# Autodesk Inventor assembly: FirstJoint
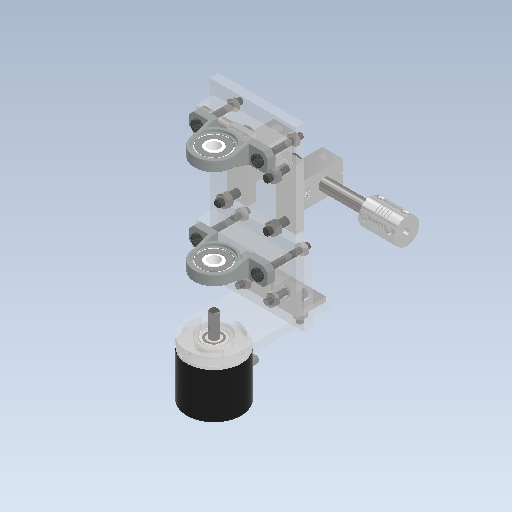
[picture p0: Inventor's stored thumbnail of the model, 512x512]
Saved by Autodesk Inventor 2021.1 (Build 251245010, 245A)
## iProperties
Created: 2023-10-30
Part Number: FirstJoint
Document SubType Name: Assembly
Designer: M
Mass: 466.393 g
Surface Area: 850.201 cm^2
Volume: 171.89 cm^3
Density: 2.71332 g/cm^3
Author: M
## Documents named in this file (17)
- F:\College\Semester_10\GP2\2DOF\2DOF_Hover\CAD\Workspaces\Workspace\FirstJoint.iam
- F:\College\Semester_10\GP2\2DOF\2DOF_Hover\CAD\Workspaces\Workspace\shaft.ipt
- F:\College\Semester_10\GP2\2DOF\2DOF_Hover\CAD\Workspaces\Workspace\Encoder.ipt
- F:\College\Semester_10\GP2\2DOF\2DOF_Hover\CAD\Workspaces\Workspace\KP008.ipt
- F:\College\Semester_10\GP2\2DOF\2DOF_Hover\CAD\Workspaces\Workspace\Holder Tube-R8.ipt
- F:\College\Semester_10\GP2\2DOF\2DOF_Hover\CAD\Workspaces\Workspace\interplate.ipt
- F:\College\Semester_10\GP2\2DOF\2DOF_Hover\CAD\Workspaces\Workspace\plateplummer.ipt
- F:\College\Semester_10\GP2\2DOF\2DOF_Hover\CAD\Workspaces\Workspace\plateencoder.ipt
- F:\College\Semester_10\GP2\2DOF\2DOF_Hover\CAD\Workspaces\Workspace\Joint1C_1.ipt
- F:\College\Semester_10\GP2\2DOF\2DOF_Hover\CAD\Workspaces\Workspace\2020RightAngle.ipt
- F:\College\Semester_10\GP2\2DOF\2DOF_Hover\CAD\Libraries\Content Center Files\en-US\ISO 4017(1)\ISO 4017 - M4 x 16 - ISO.ipt
- F:\College\Semester_10\GP2\2DOF\2DOF_Hover\CAD\Libraries\Content Center Files\en-US\ISO 4032(2)\ISO 4032 - M4 - ISO.ipt
- F:\College\Semester_10\GP2\2DOF\2DOF_Hover\CAD\Libraries\Content Center Files\en-US\ISO 7045  H\ISO 7045 - M5 x 20 - 4.8 - H - ISO.ipt
- F:\College\Semester_10\GP2\2DOF\2DOF_Hover\CAD\Libraries\Content Center Files\en-US\ISO 4032(2)\ISO 4032 - M5 - ISO.ipt
- F:\College\Semester_10\GP2\2DOF\2DOF_Hover\CAD\Libraries\Content Center Files\en-US\ISO 7045  H\ISO 7045 - M4 x 35 - 4.8 - H - ISO.ipt
- F:\College\Semester_10\GP2\2DOF\2DOF_Hover\CAD\Libraries\Content Center Files\en-US\ISO 7045  H\ISO 7045 - M4 x 30 - 4.8 - H - ISO.ipt
- F:\College\Semester_10\GP2\2DOF\2DOF_Hover\CAD\Workspaces\Workspace\Coupler_5x8.ipt
## Components (38 placed, 16 different names)
1. shaft:1 — Mate:81, Mate:82
2. Encoder:1 — Mate:17, Mate:23
3. KP008:1 — Mate:71, Mate:72, Mate:73, Mate:75, Mate:76
4. KP008:2 — Mate:18, Mate:63, Mate:64, Mate:65, Mate:67, Mate:68
5. Holder Tube-R8:1 — Mate:47, Mate:48, Mate:49, Mate:59, Mate:60
6. Holder Tube-R8:2 — Mate:51, Mate:52, Mate:55, Mate:56, Mate:79, Mate:80
7. interplate:1 — Flush:13, Mate:19, Mate:20, Mate:21, Mate:22, Angle:1, Mate:26, Mate:27, Mate:50, Mate:54, Mate:58, Mate:61, Mate:74, Mate:77
8. plateplummer:1 — Mate:19, Mate:20
9. plateplummer:2 — Mate:18, Mate:21, Mate:22
10. plateencoder:1 — Mate:26, Mate:27, Mate:28, Mate:29, Flush:14, Flush:15, Mate:39, Mate:41, Mate:42, Mate:43, Mate:45, Mate:66, Mate:70
11. Joint1C_1:1 — Mate:17, Mate:23, Angle:1, Mate:30, Flush:16, Flush:17, Mate:31, Mate:33, Mate:34, Mate:35, Mate:38
12. 2020RightAngle:1 — Mate:29, Flush:14, Mate:30, Flush:16, Mate:32, Mate:40
13. 2020RightAngle:2 — Mate:28, Flush:15, Flush:17, Mate:36, Mate:44
14. Coupler_5x8:1 — Mate:81, Mate:82
15. ISO 4017 M4 x 16:1 — Mate:31, Mate:32
16. ISO 4032 M4:1 — Mate:33, Mate:34
17. ISO 4017 M4 x 16:2 — Mate:35, Mate:36, Mate:37
18. ISO 4032 M4:2 — Mate:37, Mate:38
19. ISO 4017 M4 x 16:3 — Mate:39, Mate:40
20. ISO 4032 M4:3 — Mate:41, Mate:42
21. ISO 4017 M4 x 16:4 — Mate:43, Mate:44, Mate:46
22. ISO 4032 M4:4 — Mate:45, Mate:46
23. ISO 7045 H M5 x 20 - 4.8 - H:1 — Mate:47, Mate:48
24. ISO 4032 M5:1 — Mate:49, Mate:50
25. ISO 7045 H M5 x 20 - 4.8 - H:2 — Mate:55, Mate:56, Mate:57
26. ISO 4032 M5:2 — Mate:57, Mate:58
27. ISO 7045 H M5 x 20 - 4.8 - H:3 — Mate:59, Mate:60, Mate:62
28. ISO 4032 M5:3 — Mate:61, Mate:62
29. ISO 7045 H M5 x 20 - 4.8 - H:4 — Mate:51, Mate:52, Mate:53
30. ISO 4032 M5:4 — Mate:53, Mate:54
31. ISO 7045 H M4 x 35 - 4.8 - H:1 — Mate:63, Mate:64
32. ISO 4032 M4:5 — Mate:65, Mate:66
33. ISO 7045 H M4 x 35 - 4.8 - H:3 — Mate:67, Mate:68, Mate:69
34. ISO 4032 M4:7 — Mate:69, Mate:70
35. ISO 7045 H M4 x 30 - 4.8 - H:1 — Mate:71, Mate:72
36. ISO 4032 M4:8 — Mate:73, Mate:74
37. ISO 7045 H M4 x 30 - 4.8 - H:2 — Mate:75, Mate:76, Mate:78
38. ISO 4032 M4:9 — Mate:77, Mate:78
## Relationships (86: Mate 74, Flush 11, Angle 1)
- [Mate]: shaft:1 ↔ Holder Tube-R8:1
- [Mate]: shaft:1 ↔ Holder Tube-R8:2
- [Flush]: Holder Tube-R8:1 ↔ Holder Tube-R8:2
- [Mate] (20 mm): Holder Tube-R8:1 ↔ Holder Tube-R8:2
- [Flush]: Holder Tube-R8:2 ↔ interplate:1
- [Flush] (-29 mm): Holder Tube-R8:1 ↔ interplate:1
- [Flush] (6 mm): Holder Tube-R8:2 ↔ interplate:1
- [Flush]: interplate:1 ↔ plateplummer:1
- [Mate]: KP008:1 ↔ plateplummer:1
- [Mate]: KP008:1 ↔ plateplummer:1
- [Mate]: KP008:1 ↔ plateplummer:1
- [Mate]: KP008:2 ↔ plateplummer:2
- [Mate]: KP008:2 ↔ plateplummer:2
- [Mate]: interplate:1 ↔ plateplummer:2
- [Mate]: Encoder:1 ↔ KP008:2
- [Flush]: interplate:1 ↔ plateencoder:1
- Flush:13 (-30 mm): interplate:1
- Mate:17: Encoder:1 ↔ Joint1C_1:1
- Mate:18: KP008:2 ↔ plateplummer:2
- Mate:19: interplate:1 ↔ plateplummer:1
- Mate:20: interplate:1 ↔ plateplummer:1
- Mate:21: interplate:1 ↔ plateplummer:2
- Mate:22: interplate:1 ↔ plateplummer:2
- Mate:23: Encoder:1 ↔ Joint1C_1:1
- Angle:1 (0 deg): interplate:1 ↔ Joint1C_1:1
- Mate:26: interplate:1 ↔ plateencoder:1
- Mate:27: interplate:1 ↔ plateencoder:1
- Mate:28: plateencoder:1 ↔ 2020RightAngle:2
- Mate:29: plateencoder:1 ↔ 2020RightAngle:1
- Flush:14: plateencoder:1 ↔ 2020RightAngle:1
- Flush:15: plateencoder:1 ↔ 2020RightAngle:2
- Mate:30: Joint1C_1:1 ↔ 2020RightAngle:1
- Flush:16: Joint1C_1:1 ↔ 2020RightAngle:1
- Flush:17: Joint1C_1:1 ↔ 2020RightAngle:2
- Mate:31: Joint1C_1:1 ↔ ISO 4017 M4 x 16:1
- Mate:32: 2020RightAngle:1 ↔ ISO 4017 M4 x 16:1
- Mate:33: Joint1C_1:1 ↔ ISO 4032 M4:1
- Mate:34: Joint1C_1:1 ↔ ISO 4032 M4:1
- Mate:35: Joint1C_1:1 ↔ ISO 4017 M4 x 16:2
- Mate:36: 2020RightAngle:2 ↔ ISO 4017 M4 x 16:2
- Mate:37: ISO 4017 M4 x 16:2 ↔ ISO 4032 M4:2
- Mate:38: Joint1C_1:1 ↔ ISO 4032 M4:2
- Mate:39: plateencoder:1 ↔ ISO 4017 M4 x 16:3
- Mate:40: 2020RightAngle:1 ↔ ISO 4017 M4 x 16:3
- Mate:41: plateencoder:1 ↔ ISO 4032 M4:3
- Mate:42: plateencoder:1 ↔ ISO 4032 M4:3
- Mate:43: plateencoder:1 ↔ ISO 4017 M4 x 16:4
- Mate:44: 2020RightAngle:2 ↔ ISO 4017 M4 x 16:4
- Mate:45: plateencoder:1 ↔ ISO 4032 M4:4
- Mate:46: ISO 4017 M4 x 16:4 ↔ ISO 4032 M4:4
- Mate:47: Holder Tube-R8:1 ↔ ISO 7045 H M5 x 20 - 4.8 - H:1
- Mate:48: Holder Tube-R8:1 ↔ ISO 7045 H M5 x 20 - 4.8 - H:1
- Mate:49: Holder Tube-R8:1 ↔ ISO 4032 M5:1
- Mate:50: interplate:1 ↔ ISO 4032 M5:1
- Mate:51: Holder Tube-R8:2 ↔ ISO 7045 H M5 x 20 - 4.8 - H:4
- Mate:52: Holder Tube-R8:2 ↔ ISO 7045 H M5 x 20 - 4.8 - H:4
- Mate:53: ISO 7045 H M5 x 20 - 4.8 - H:4 ↔ ISO 4032 M5:4
- Mate:54: interplate:1 ↔ ISO 4032 M5:4
- Mate:55: Holder Tube-R8:2 ↔ ISO 7045 H M5 x 20 - 4.8 - H:2
- Mate:56: Holder Tube-R8:2 ↔ ISO 7045 H M5 x 20 - 4.8 - H:2
- Mate:57: ISO 7045 H M5 x 20 - 4.8 - H:2 ↔ ISO 4032 M5:2
- Mate:58: interplate:1 ↔ ISO 4032 M5:2
- Mate:59: Holder Tube-R8:1 ↔ ISO 7045 H M5 x 20 - 4.8 - H:3
- Mate:60: Holder Tube-R8:1 ↔ ISO 7045 H M5 x 20 - 4.8 - H:3
- Mate:61: interplate:1 ↔ ISO 4032 M5:3
- Mate:62: ISO 7045 H M5 x 20 - 4.8 - H:3 ↔ ISO 4032 M5:3
- Mate:63: KP008:2 ↔ ISO 7045 H M4 x 35 - 4.8 - H:1
- Mate:64: KP008:2 ↔ ISO 7045 H M4 x 35 - 4.8 - H:1
- Mate:65: KP008:2 ↔ ISO 4032 M4:5
- Mate:66: plateencoder:1 ↔ ISO 4032 M4:5
- Mate:67: KP008:2 ↔ ISO 7045 H M4 x 35 - 4.8 - H:3
- Mate:68: KP008:2 ↔ ISO 7045 H M4 x 35 - 4.8 - H:3
- Mate:69: ISO 7045 H M4 x 35 - 4.8 - H:3 ↔ ISO 4032 M4:7
- Mate:70: plateencoder:1 ↔ ISO 4032 M4:7
- Mate:71: KP008:1 ↔ ISO 7045 H M4 x 30 - 4.8 - H:1
- Mate:72: KP008:1 ↔ ISO 7045 H M4 x 30 - 4.8 - H:1
- Mate:73: KP008:1 ↔ ISO 4032 M4:8
- Mate:74: interplate:1 ↔ ISO 4032 M4:8
- Mate:75: KP008:1 ↔ ISO 7045 H M4 x 30 - 4.8 - H:2
- Mate:76: KP008:1 ↔ ISO 7045 H M4 x 30 - 4.8 - H:2
- Mate:77: interplate:1 ↔ ISO 4032 M4:9
- Mate:78: ISO 7045 H M4 x 30 - 4.8 - H:2 ↔ ISO 4032 M4:9
- Mate:79 (-9 mm): Holder Tube-R8:2
- Mate:80: Holder Tube-R8:2
- Mate:81: shaft:1 ↔ Coupler_5x8:1
- Mate:82 (-12 mm): shaft:1 ↔ Coupler_5x8:1
